# Autodesk Inventor assembly: Entry solid wood Facade
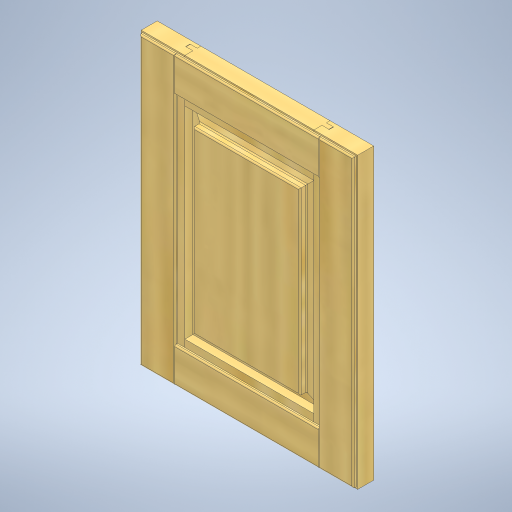
[picture p0: Inventor's stored thumbnail of the model, 512x512]
Saved by Autodesk Inventor 2024 (Build 280153000, 153)
## iProperties
Created: 2014-03-21
Part Number: Entry solid wood Facade
Document SubType Name: Assembly
Designer: SauliusD
Description: Entry solid wood door
Author: SauliusD
## Documents named in this file (7)
- C:\W4INV 2024 Design\iBOX LIBRARY\Facades\Entry solid wood\Entry solid wood Facade.iam
- C:\W4INV 2024 Design\iBOX LIBRARY\Facades\Entry solid wood\Facade Right Frame.ipt
- C:\W4INV 2024 Design\iBOX LIBRARY\Facades\Entry solid wood\Facade Left Frame.ipt
- C:\W4INV 2024 Design\iBOX LIBRARY\Facades\Entry solid wood\Facade Bottom Frame.ipt
- C:\W4INV 2024 Design\iBOX LIBRARY\Facades\Entry solid wood\Facade Top Frame.ipt
- C:\W4INV 2024 Design\iBOX LIBRARY\Facades\Entry solid wood\Facade Board.ipt
- C:\W4INV 2024 Design\iBOX LIBRARY\Facades\Entry solid wood\Entry solid wood facade.ipt
## Components (6 placed, 6 different names)
1. @Skeleton — Flush:19, Flush:20, Flush:21
2. Facade Board:1 — Flush:16, Flush:17, Flush:18
3. Facade Top Frame:1 — Flush:13, Flush:14, Flush:15
4. Facade Bottom Frame:1 — Flush:10, Flush:11, Flush:12
5. Facade Left Frame:1 — Flush:7, Flush:8, Flush:9
6. Facade Right Frame:1 — Flush:4, Flush:5, Flush:6
## Relationships (18: Flush 18)
- Flush:4: Facade Right Frame:1
- Flush:5: Facade Right Frame:1
- Flush:6: Facade Right Frame:1
- Flush:7: Facade Left Frame:1
- Flush:8: Facade Left Frame:1
- Flush:9: Facade Left Frame:1
- Flush:10: Facade Bottom Frame:1
- Flush:11: Facade Bottom Frame:1
- Flush:12: Facade Bottom Frame:1
- Flush:13: Facade Top Frame:1
- Flush:14: Facade Top Frame:1
- Flush:15: Facade Top Frame:1
- Flush:16: Facade Board:1
- Flush:17: Facade Board:1
- Flush:18: Facade Board:1
- Flush:19: @Skeleton
- Flush:20: @Skeleton
- Flush:21: @Skeleton
